# Autodesk Inventor assembly: SensorAssembly
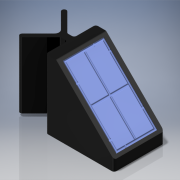
[picture p0: Inventor's stored thumbnail of the model, 180x180]
Saved by Autodesk Inventor 2019 (Build 230136000, 136)
## iProperties
Created: 2018-09-02
Part Number: SensorAssembly
Document SubType Name: Assembly
Designer: Crater-Windows
Author: Crater-Windows
## Documents named in this file (4)
- C:\Users\Crater-Windows\Google Drive\Academics\William Jewell College\Extracurricular\Honors Project - DROP\DROP - Sensor Housing\SensorAssembly.iam
- C:\Users\Crater-Windows\Google Drive\Academics\William Jewell College\Extracurricular\Honors Project - DROP\DROP - Sensor Housing\MainHousing.ipt
- C:\Users\Crater-Windows\Google Drive\Academics\William Jewell College\Extracurricular\Honors Project - DROP\DROP - Sensor Housing\SolarPanel.ipt
- C:\Users\Crater-Windows\Google Drive\Academics\William Jewell College\Extracurricular\Honors Project - DROP\DROP - Sensor Housing\MainHousing_BottomPlate.ipt
## Components (3 placed, 3 different names)
1. MainHousing:1 — Mate:1, Mate:2, Mate:3, Insert:1, Flush:1, Mate:4, Flush:2
2. SolarPanel:1 — Mate:1, Mate:2, Mate:3
3. MainHousing_BottomPlate:1 — Insert:1, Flush:1, Mate:4, Flush:2
## Relationships (7: Mate 4, Flush 2, Insert 1)
- Mate:1: MainHousing:1 ↔ SolarPanel:1
- Mate:2: MainHousing:1 ↔ SolarPanel:1
- Mate:3: MainHousing:1 ↔ SolarPanel:1
- Insert:1: MainHousing:1 ↔ MainHousing_BottomPlate:1
- Flush:1: MainHousing:1 ↔ MainHousing_BottomPlate:1
- Mate:4: MainHousing:1 ↔ MainHousing_BottomPlate:1
- Flush:2: MainHousing:1 ↔ MainHousing_BottomPlate:1
